# Autodesk Inventor assembly: Samolot bez sparow
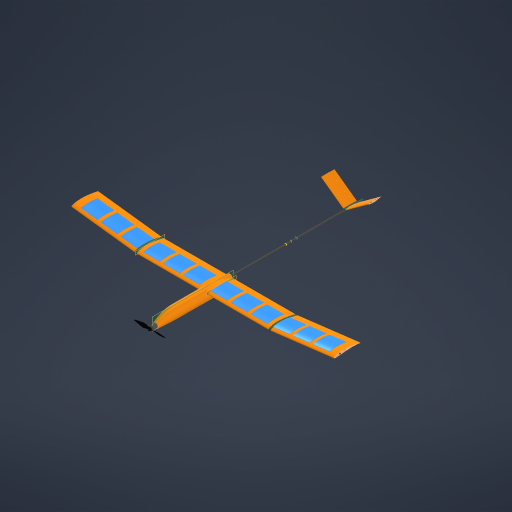
[picture p0: Inventor's stored thumbnail of the model, 512x512]
Saved by Autodesk Inventor 2023 (Build 270158000, 158)
## iProperties
Created: 2023-01-05
Part Number: Samolot bez sparow
Document SubType Name: Assembly
Designer: szykr
Author: szykr
## Documents named in this file (11)
- D:\Folder Instalacyjny\GitHub Pliki\Solaris\new model\Samolot bez sparow.iam
- D:\Folder Instalacyjny\GitHub Pliki\Solaris\new model\Skrzydło.iam
- D:\Folder Instalacyjny\GitHub Pliki\Solaris\new model\Tail\Tail.iam
- D:\Folder Instalacyjny\GitHub Pliki\Solaris\new model\nowy kadłub.ipt
- D:\Folder Instalacyjny\GitHub Pliki\Solaris\new model\Poszycie.ipt
- D:\Folder Instalacyjny\GitHub Pliki\Solaris\new model\Tail\Poszycie skrzydlo glowne.ipt
- D:\Folder Instalacyjny\GitHub Pliki\Solaris\new model\Poszycie skrzydlo glowne.ipt
- D:\Folder Instalacyjny\GitHub Pliki\Solaris\new model\Poszycie skrzydlo sterowe.ipt
- D:\Folder Instalacyjny\GitHub Pliki\Solaris\new model\Silnik.ipt
- D:\Folder Instalacyjny\GitHub Pliki\Solaris\new model\APC_9x6.ipt
- D:\Folder Instalacyjny\GitHub Pliki\Solaris\new model\Panele.ipt
## Components (22 placed, 9 different names)
1. Tail:1 [sub-assembly] — Insert:1
2. nowy kadłub:1 — Mate:1, Mate:2, Mate:3, Insert:1, Mate:4, Mate:5, Angle:1, Flush:6
3. Skrzydło:1 [sub-assembly] — Mate:1, Mate:2, Mate:3, Flush:1, Flush:2, Mate:6, Mate:7, Flush:3, Flush:4, Mate:8, Mate:9, Flush:5, Mate:10, Mate:11, Flush:8, Mate:12, Mate:13, Mate:14, Mate:15
4. Poszycie:1 — Mate:4, Mate:5, Angle:1
5. Poszycie skrzydlo glowne:1 — Flush:1, Flush:2
6. Poszycie skrzydlo glowne:2 — Mate:6, Mate:7, Flush:3, Flush:7
7. Poszycie skrzydlo sterowe:1 — Flush:4, Flush:9
8. Poszycie skrzydlo sterowe:2 — Mate:8, Mate:9, Flush:5, Flush:10
9. Silnik:1 — Flush:6, Insert:2
10. APC_9x6:1 — Insert:2
11. Panele:1 — Flush:7
12. Panele:2
13. Panele:3
14. Panele:4 — Mate:10, Mate:11, Flush:8
15. Panele:5
16. Panele:6
17. Panele:7 — Mate:12, Mate:13, Flush:9
18. Panele:8
19. Panele:9
20. Panele:10 — Mate:14, Mate:15, Flush:10
21. Panele:11
22. Panele:12
## Component patterns: (3 elements, first: Panele:1), (3 elements, first: Panele:4), (3 elements, first: Panele:7), (3 elements, first: Panele:10)
## Relationships (28: Mate 15, Flush 10, Insert 2, Angle 1)
- Mate:1: nowy kadłub:1 ↔ Skrzydło:1
- Mate:2: nowy kadłub:1 ↔ Skrzydło:1
- Mate:3: nowy kadłub:1 ↔ Skrzydło:1
- Insert:1 (-40 mm): Tail:1 ↔ nowy kadłub:1
- Mate:4: nowy kadłub:1 ↔ Poszycie:1
- Mate:5: nowy kadłub:1 ↔ Poszycie:1
- Angle:1 (180 deg): nowy kadłub:1 ↔ Poszycie:1
- Flush:1: Skrzydło:1 ↔ Poszycie skrzydlo glowne:1
- Flush:2: Skrzydło:1 ↔ Poszycie skrzydlo glowne:1
- Mate:6: Skrzydło:1 ↔ Poszycie skrzydlo glowne:2
- Mate:7: Skrzydło:1 ↔ Poszycie skrzydlo glowne:2
- Flush:3: Skrzydło:1 ↔ Poszycie skrzydlo glowne:2
- Flush:4: Skrzydło:1 ↔ Poszycie skrzydlo sterowe:1
- Mate:8: Skrzydło:1 ↔ Poszycie skrzydlo sterowe:2
- Mate:9: Skrzydło:1 ↔ Poszycie skrzydlo sterowe:2
- Flush:5: Skrzydło:1 ↔ Poszycie skrzydlo sterowe:2
- Flush:6: nowy kadłub:1 ↔ Silnik:1
- Insert:2: Silnik:1 ↔ APC_9x6:1
- Flush:7: Poszycie skrzydlo glowne:2 ↔ Panele:1
- Mate:10: Skrzydło:1 ↔ Panele:4
- Mate:11: Skrzydło:1 ↔ Panele:4
- Flush:8: Skrzydło:1 ↔ Panele:4
- Mate:12: Skrzydło:1 ↔ Panele:7
- Mate:13: Skrzydło:1 ↔ Panele:7
- Flush:9: Poszycie skrzydlo sterowe:1 ↔ Panele:7
- Mate:14: Skrzydło:1 ↔ Panele:10
- Mate:15: Skrzydło:1 ↔ Panele:10
- Flush:10: Poszycie skrzydlo sterowe:2 ↔ Panele:10
